# Autodesk Inventor assembly: New_Odom_Assembly
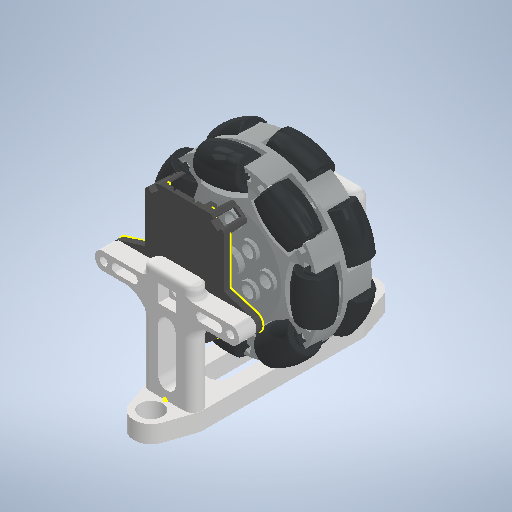
[picture p0: Inventor's stored thumbnail of the model, 512x512]
Saved by Autodesk Inventor 2025.1 (Build 291241020, 241B)
## iProperties
Created: 2024-11-18
Part Number: New_Odom_Assembly
Document SubType Name: Assembly
Designer: AtuStem
Author: AtuStem
## Documents named in this file (4)
- C:\Users\AtuStem\Documents\GitHub\ATUM-V5RC-High-Stakes-CAD\Odometers_Collin\New_Odom_Assembly.iam
- C:\Users\AtuStem\Documents\GitHub\ATUM-V5RC-High-Stakes-CAD\Odometers_Collin\IQ_OMNI.iam
- C:\Users\AtuStem\Documents\GitHub\ATUM-V5RC-High-Stakes-CAD\Latest_Odom.ipt
- C:\Users\AtuStem\Documents\GitHub\ATUM-V5RC-High-Stakes-CAD\Odometers_Collin\Encoder_Base.ipt
## Components (3 placed, 3 different names)
1. IQ_OMNI:1 [sub-assembly] — Mate:1
2. Latest_Odom:1 — Mate:1, Mate:2, Mate:3, Mate:4
3. Encoder_Base:1 — Mate:2, Mate:3, Mate:4
## Relationships (4: Mate 4)
- Mate:1: IQ_OMNI:1 ↔ Latest_Odom:1
- Mate:2: Latest_Odom:1 ↔ Encoder_Base:1
- Mate:3: Latest_Odom:1 ↔ Encoder_Base:1
- Mate:4: Latest_Odom:1 ↔ Encoder_Base:1
